# Autodesk Inventor assembly: Ball Field
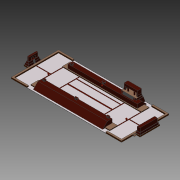
[picture p0: Inventor's stored thumbnail of the model, 180x180]
Saved by Autodesk Inventor 2015 (Build 190159000, 159)
## iProperties
Created: 2016-12-01
Part Number: Ball Field
Document SubType Name: Assembly
Designer: Simms
Author: Simms
## Documents named in this file (7)
- C:\Users\Simms\Documents\Inventor\MuseumCAP\Ball Field.iam
- C:\Users\Simms\Documents\Inventor\MuseumCAP\Ball Field.ipt
- C:\Users\Simms\Documents\Inventor\MuseumCAP\Wall Hoop.ipt
- C:\Users\Simms\Documents\Inventor\MuseumCAP\Floor Goal.ipt
- C:\Users\Simms\Documents\Inventor\MuseumCAP\Side1.ipt
- C:\Users\Simms\Documents\Inventor\MuseumCAP\Side2.ipt
- C:\Users\Simms\Documents\Inventor\MuseumCAP\Stand.ipt
## Components (8 placed, 6 different names)
1. Ball Field:1 — Mate:1, Flush:1, Flush:2, Mate:2, Flush:3, Flush:4, Mate:3, Flush:5, Mate:4, Flush:6, Mate:5, Flush:7, Flush:8, Mate:6, Flush:9, Flush:10, Mate:7, Flush:11, Flush:12
2. Wall Hoop:1 — Mate:1, Flush:1, Flush:2
3. Wall Hoop:2 — Mate:2, Flush:3, Flush:4
4. Floor Goal:1 — Mate:4, Flush:6
5. Floor Goal:2 — Mate:3, Flush:5
6. Side1:1 — Mate:5, Flush:7, Flush:8
7. Side2:1 — Mate:6, Flush:9, Flush:10
8. Stand:1 — Mate:7, Flush:11, Flush:12
## Relationships (19: Flush 12, Mate 7)
- Mate:1: Ball Field:1 ↔ Wall Hoop:1
- Flush:1 (-6.35 mm): Ball Field:1 ↔ Wall Hoop:1
- Flush:2 (-555.625 mm): Ball Field:1 ↔ Wall Hoop:1
- Mate:2: Ball Field:1 ↔ Wall Hoop:2
- Flush:3 (555.625 mm): Ball Field:1 ↔ Wall Hoop:2
- Flush:4 (6.35 mm): Ball Field:1 ↔ Wall Hoop:2
- Mate:3: Ball Field:1 ↔ Floor Goal:2
- Flush:5: Ball Field:1 ↔ Floor Goal:2
- Mate:4: Ball Field:1 ↔ Floor Goal:1
- Flush:6: Ball Field:1 ↔ Floor Goal:1
- Mate:5: Ball Field:1 ↔ Side1:1
- Flush:7 (28.575 mm): Ball Field:1 ↔ Side1:1
- Flush:8 (28.575 mm): Ball Field:1 ↔ Side1:1
- Mate:6: Ball Field:1 ↔ Side2:1
- Flush:9 (19.05 mm): Ball Field:1 ↔ Side2:1
- Flush:10 (19.05 mm): Ball Field:1 ↔ Side2:1
- Mate:7: Ball Field:1 ↔ Stand:1
- Flush:11 (17.2412 mm): Ball Field:1 ↔ Stand:1
- Flush:12 (-42.164 mm): Ball Field:1 ↔ Stand:1
